# Autodesk Inventor assembly: xtion_custom_assembly_v2
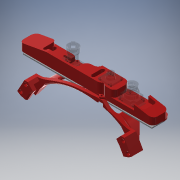
[picture p0: Inventor's stored thumbnail of the model, 180x180]
Saved by Autodesk Inventor 2017 (Build 210142000, 142)
## iProperties
Created: 2016-11-28
Part Number: xtion_custom_assembly_v2
Document SubType Name: Assembly
Designer: Ali
Author: Ali
## Documents named in this file (7)
- C:\Users\Alistair\Dropbox\Work\HeadSLAM\prototype-2\xtion_custom_assembly_v2.iam
- C:\Users\Alistair\Dropbox\Work\HeadSLAM\prototype-2\head_mount_v2.ipt
- C:\Users\Alistair\Dropbox\Work\HeadSLAM\xtion-internal\xtion_mainboard.ipt
- C:\Users\Alistair\Dropbox\Work\HeadSLAM\prototype-2\xtion_custom_v2.ipt
- C:\Users\Alistair\Dropbox\Work\HeadSLAM\xtion-internal\xtion_ir_cam.ipt
- C:\Users\Alistair\Dropbox\Work\HeadSLAM\xtion-internal\xtion_projector.ipt
- C:\Users\Alistair\Dropbox\Work\HeadSLAM\xtion-internal\xtion_rgb_cam.ipt
## Components (6 placed, 6 different names)
1. head_mount_v2:1 — Rigid:1, Rigid:5
2. xtion_mainboard:1 — Rigid:1
3. xtion_custom_v2:1 — Rigid:2, Rigid:3, Rigid:4, Rigid:5
4. xtion_ir_cam:1 — Rigid:2
5. xtion_projector:1 — Rigid:4
6. xtion_rgb_cam:1 — Rigid:3
## Relationships (5: WeldJoint 5)
- Rigid:1 [WeldJoint]: head_mount_v2:1 ↔ xtion_mainboard:1
- Rigid:2 [WeldJoint]: xtion_custom_v2:1 ↔ xtion_ir_cam:1
- Rigid:3 [WeldJoint]: xtion_custom_v2:1 ↔ xtion_rgb_cam:1
- Rigid:4 [WeldJoint]: xtion_custom_v2:1 ↔ xtion_projector:1
- Rigid:5 [WeldJoint]: head_mount_v2:1 ↔ xtion_custom_v2:1
